# Autodesk Inventor assembly: Stewart-Body-KST-DS215
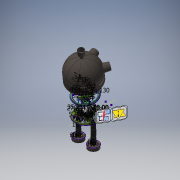
[picture p0: Inventor's stored thumbnail of the model, 180x180]
Saved by Autodesk Inventor 2018.2 (Build 222227000, 227)
## iProperties
Created: 2018-02-24
Part Number: Stewart-Body-KST-DS215
Material: Generisch
Document SubType Name: Assembly
Designer: JochenAlt
Author: JochenAlt
## Documents named in this file (11)
- D:\Projects\Donna\CAD\Donna.iam
- D:\Projects\Donna\CAD\Stewart-Base.iam
- D:\Projects\Donna\CAD\Body-Rod.iam
- D:\Projects\Donna\CAD\Stewart-Body.iam
- D:\Projects\Donna\CAD\Servo-Arm-Head-20mm-Ball-Joint.iam
- D:\Projects\Donna\CAD\Stewart-Head.iam
- D:\Projects\Donna\CAD\Head-Rod.iam
- D:\Projects\Donna\CAD\Donnas Head.ipt
- D:\Projects\Donna\CAD\Leg-Part.ipt
- D:\Projects\Donna\CAD\LegScrew.ipt
- D:\Projects\Donna\CAD\Foot.ipt
## Components (38 placed, 9 different names)
1. Stewart-Body:1 [sub-assembly] — Passend:80, Passend:81, Passend:82, Passend:83, Passend:84, Passend:85, Passend:87, Passend:89, Passend:90, Passend:91, Passend:94, Passend:97, Passend:106, Passend:107, Passend:108, Passend:109, Passend:112
2. BodyRod:1 [sub-assembly] — Passend:21, Passend:95
3. BodyRod:2 [sub-assembly] — Passend:22, Passend:96
4. BodyRod:3 [sub-assembly] — Passend:23, Passend:88
5. BodyRod:4 [sub-assembly] — Passend:24, Passend:86
6. BodyRod:5 [sub-assembly] — Passend:19, Passend:93
7. BodyRod:6 [sub-assembly] — Passend:20, Passend:92
8. Stewart-Body-KST215MG:1 [sub-assembly] — Passend:19, Passend:20, Passend:21, Passend:22, Passend:23, Passend:24, Passend:49, Passend:50, Passend:51, Passend:52, Passend:53, Passend:54, Passend:72, Passend:73, Passend:74, Passend:75, Passend:76, Passend:77
9. Servo-Arm-Head-20mm-Ball-Joint:1 [sub-assembly] — Passend:39, Passend:49, Passend:73
10. Servo-Arm-Head-20mm-Ball-Joint:2 [sub-assembly] — Passend:40, Passend:50, Passend:72
11. Servo-Arm-Head-20mm-Ball-Joint:3 [sub-assembly] — Passend:42, Passend:54, Passend:76
12. Servo-Arm-Head-20mm-Ball-Joint:4 [sub-assembly] — Passend:41, Passend:53, Passend:77
13. Servo-Arm-Head-20mm-Ball-Joint:5 [sub-assembly] — Passend:37, Passend:52, Passend:74
14. Servo-Arm-Head-20mm-Ball-Joint:6 [sub-assembly] — Passend:38, Passend:51, Passend:75
15. Stewart-Head:1 [sub-assembly] — Passend:43, Passend:44, Passend:45, Passend:46, Passend:47, Passend:48, Passend:118, Passend:119, Winkel:1
16. BodyRod:7 [sub-assembly] — Passend:39, Passend:43
17. BodyRod:8 [sub-assembly] — Passend:40, Passend:44
18. BodyRod:9 [sub-assembly] — Passend:41, Passend:47
19. BodyRod:10 [sub-assembly] — Passend:42, Passend:48
20. BodyRod:11 [sub-assembly] — Passend:38, Passend:46
21. BodyRod:12 [sub-assembly] — Passend:37, Passend:45
22. Donnas Head:1 — Passend:118, Passend:119, Winkel:1
23. Servo-Arm-Head-20mm-Ball-Joint:7 [sub-assembly] — Passend:80, Passend:87, Passend:88
24. Servo-Arm-Head-20mm-Ball-Joint:8 [sub-assembly] — Passend:82, Passend:94, Passend:95
25. Servo-Arm-Head-20mm-Ball-Joint:9 [sub-assembly] — Passend:83, Passend:91, Passend:93
26. Servo-Arm-Head-20mm-Ball-Joint:10 [sub-assembly] — Passend:84, Passend:85, Passend:86
27. Servo-Arm-Head-20mm-Ball-Joint:11 [sub-assembly] — Passend:89, Passend:90, Passend:92
28. Servo-Arm-Head-20mm-Ball-Joint:12 [sub-assembly] — Passend:81, Passend:96, Passend:97
29. Leg-Part:1 — Passend:102, Passend:104, Passend:110, Passend:112
30. Leg-Part:2 — Passend:102, Passend:103, Passend:105, Passend:116, Passend:120
31. Leg-Part:3 — Passend:103, Passend:104, Passend:105
32. Leg-Part:4 — Passend:99, Passend:101, Passend:117, Passend:121
33. Leg-Part:5 — Passend:98, Passend:100, Passend:111, Passend:113
34. Leg-Part:6 — Passend:98, Passend:99, Passend:100, Passend:101
35. LegScrew:1 — Passend:106, Passend:109, Passend:110
36. LegScrew:2 — Passend:107, Passend:108, Passend:111, Passend:113
37. Foot:1 — Passend:117, Passend:121
38. Foot:2 — Passend:116, Passend:120
## Relationships (71: Mate 70, Angle 1)
- Passend:19 [Mate]: BodyRod:5 ↔ Stewart-Body-KST215MG:1
- Passend:20 [Mate]: BodyRod:6 ↔ Stewart-Body-KST215MG:1
- Passend:21 [Mate]: BodyRod:1 ↔ Stewart-Body-KST215MG:1
- Passend:22 [Mate]: BodyRod:2 ↔ Stewart-Body-KST215MG:1
- Passend:23 [Mate]: BodyRod:3 ↔ Stewart-Body-KST215MG:1
- Passend:24 [Mate]: BodyRod:4 ↔ Stewart-Body-KST215MG:1
- Passend:37 [Mate]: Servo-Arm-Head-20mm-Ball-Joint:5 ↔ BodyRod:12
- Passend:38 [Mate]: Servo-Arm-Head-20mm-Ball-Joint:6 ↔ BodyRod:11
- Passend:39 [Mate]: Servo-Arm-Head-20mm-Ball-Joint:1 ↔ BodyRod:7
- Passend:40 [Mate]: Servo-Arm-Head-20mm-Ball-Joint:2 ↔ BodyRod:8
- Passend:41 [Mate]: Servo-Arm-Head-20mm-Ball-Joint:4 ↔ BodyRod:9
- Passend:42 [Mate]: Servo-Arm-Head-20mm-Ball-Joint:3 ↔ BodyRod:10
- Passend:43 [Mate]: Stewart-Head:1 ↔ BodyRod:7
- Passend:44 [Mate]: Stewart-Head:1 ↔ BodyRod:8
- Passend:45 [Mate]: Stewart-Head:1 ↔ BodyRod:12
- Passend:46 [Mate]: Stewart-Head:1 ↔ BodyRod:11
- Passend:47 [Mate]: Stewart-Head:1 ↔ BodyRod:9
- Passend:48 [Mate]: Stewart-Head:1 ↔ BodyRod:10
- Passend:49 [Mate]: Stewart-Body-KST215MG:1 ↔ Servo-Arm-Head-20mm-Ball-Joint:1
- Passend:50 [Mate]: Stewart-Body-KST215MG:1 ↔ Servo-Arm-Head-20mm-Ball-Joint:2
- Passend:51 [Mate]: Stewart-Body-KST215MG:1 ↔ Servo-Arm-Head-20mm-Ball-Joint:6
- Passend:52 [Mate]: Stewart-Body-KST215MG:1 ↔ Servo-Arm-Head-20mm-Ball-Joint:5
- Passend:53 [Mate]: Stewart-Body-KST215MG:1 ↔ Servo-Arm-Head-20mm-Ball-Joint:4
- Passend:54 [Mate]: Stewart-Body-KST215MG:1 ↔ Servo-Arm-Head-20mm-Ball-Joint:3
- Passend:72 [Mate]: Stewart-Body-KST215MG:1 ↔ Servo-Arm-Head-20mm-Ball-Joint:2
- Passend:73 [Mate]: Stewart-Body-KST215MG:1 ↔ Servo-Arm-Head-20mm-Ball-Joint:1
- Passend:74 [Mate]: Stewart-Body-KST215MG:1 ↔ Servo-Arm-Head-20mm-Ball-Joint:5
- Passend:75 [Mate]: Stewart-Body-KST215MG:1 ↔ Servo-Arm-Head-20mm-Ball-Joint:6
- Passend:76 [Mate]: Stewart-Body-KST215MG:1 ↔ Servo-Arm-Head-20mm-Ball-Joint:3
- Passend:77 [Mate]: Stewart-Body-KST215MG:1 ↔ Servo-Arm-Head-20mm-Ball-Joint:4
- Passend:80 [Mate]: Stewart-Body:1 ↔ Servo-Arm-Head-20mm-Ball-Joint:7
- Passend:81 [Mate]: Stewart-Body:1 ↔ Servo-Arm-Head-20mm-Ball-Joint:12
- Passend:82 [Mate]: Stewart-Body:1 ↔ Servo-Arm-Head-20mm-Ball-Joint:8
- Passend:83 [Mate]: Stewart-Body:1 ↔ Servo-Arm-Head-20mm-Ball-Joint:9
- Passend:84 [Mate]: Stewart-Body:1 ↔ Servo-Arm-Head-20mm-Ball-Joint:10
- Passend:85 [Mate]: Stewart-Body:1 ↔ Servo-Arm-Head-20mm-Ball-Joint:10
- Passend:86 [Mate]: BodyRod:4 ↔ Servo-Arm-Head-20mm-Ball-Joint:10
- Passend:87 [Mate]: Stewart-Body:1 ↔ Servo-Arm-Head-20mm-Ball-Joint:7
- Passend:88 [Mate]: BodyRod:3 ↔ Servo-Arm-Head-20mm-Ball-Joint:7
- Passend:89 [Mate]: Stewart-Body:1 ↔ Servo-Arm-Head-20mm-Ball-Joint:11
- Passend:90 [Mate]: Stewart-Body:1 ↔ Servo-Arm-Head-20mm-Ball-Joint:11
- Passend:91 [Mate]: Stewart-Body:1 ↔ Servo-Arm-Head-20mm-Ball-Joint:9
- Passend:92 [Mate]: BodyRod:6 ↔ Servo-Arm-Head-20mm-Ball-Joint:11
- Passend:93 [Mate]: BodyRod:5 ↔ Servo-Arm-Head-20mm-Ball-Joint:9
- Passend:94 [Mate]: Stewart-Body:1 ↔ Servo-Arm-Head-20mm-Ball-Joint:8
- Passend:95 [Mate]: BodyRod:1 ↔ Servo-Arm-Head-20mm-Ball-Joint:8
- Passend:96 [Mate]: BodyRod:2 ↔ Servo-Arm-Head-20mm-Ball-Joint:12
- Passend:97 [Mate]: Stewart-Body:1 ↔ Servo-Arm-Head-20mm-Ball-Joint:12
- Passend:98 [Mate]: Leg-Part:5 ↔ Leg-Part:6
- Passend:99 [Mate]: Leg-Part:4 ↔ Leg-Part:6
- Passend:100 [Mate]: Leg-Part:5 ↔ Leg-Part:6
- Passend:101 [Mate]: Leg-Part:4 ↔ Leg-Part:6
- Passend:102 [Mate]: Leg-Part:1 ↔ Leg-Part:2
- Passend:103 [Mate]: Leg-Part:2 ↔ Leg-Part:3
- Passend:104 [Mate]: Leg-Part:1 ↔ Leg-Part:3
- Passend:105 [Mate]: Leg-Part:2 ↔ Leg-Part:3
- Passend:106 [Mate]: Stewart-Body:1 ↔ LegScrew:1
- Passend:107 [Mate]: Stewart-Body:1 ↔ LegScrew:2
- Passend:108 [Mate]: Stewart-Body:1 ↔ LegScrew:2
- Passend:109 [Mate]: Stewart-Body:1 ↔ LegScrew:1
- Passend:110 [Mate]: Leg-Part:1 ↔ LegScrew:1
- Passend:111 [Mate]: Leg-Part:5 ↔ LegScrew:2
- Passend:112 [Mate]: Stewart-Body:1 ↔ Leg-Part:1
- Passend:113 [Mate]: Leg-Part:5 ↔ LegScrew:2
- Passend:116 [Mate]: Leg-Part:2 ↔ Foot:2
- Passend:117 [Mate]: Leg-Part:4 ↔ Foot:1
- Passend:118 [Mate]: Stewart-Head:1 ↔ Donnas Head:1
- Passend:119 [Mate]: Stewart-Head:1 ↔ Donnas Head:1
- Passend:120 [Mate]: Leg-Part:2 ↔ Foot:2
- Passend:121 [Mate]: Leg-Part:4 ↔ Foot:1
- Winkel:1 [Angle] (0 deg): Stewart-Head:1 ↔ Donnas Head:1
